# Autodesk Inventor assembly: Scoreboard
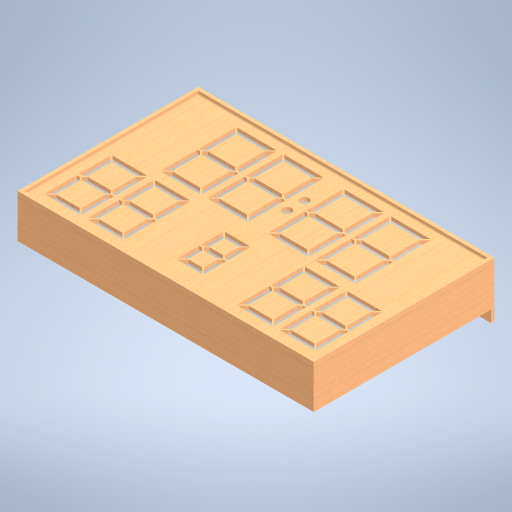
[picture p0: Inventor's stored thumbnail of the model, 512x512]
Saved by Autodesk Inventor 2024 (Build 280153000, 153)
## iProperties
Created: 2024-02-15
Part Number: Scoreboard
Document SubType Name: Assembly
Designer: haniv
Author: haniv
## Documents named in this file (8)
- C:\Users\haniv\Desktop\Unterlagen\Projekte\7_Segment_Anzeige\ScoreDisplay\CAD\Scoreboard.iam
- C:\Users\haniv\Desktop\Unterlagen\Projekte\7_Segment_Anzeige\ScoreDisplay\CAD\Components\Aluminium_Grundplatte.ipt
- C:\Users\haniv\Desktop\Unterlagen\Projekte\7_Segment_Anzeige\ScoreDisplay\CAD\Components\MDF_Anzeige.ipt
- C:\Users\haniv\Desktop\Unterlagen\Projekte\7_Segment_Anzeige\ScoreDisplay\CAD\Components\Längsseite_Gehäuse.ipt
- C:\Users\haniv\Desktop\Unterlagen\Projekte\7_Segment_Anzeige\ScoreDisplay\CAD\Components\Querseite_Gehäuse.ipt
- C:\Users\haniv\Desktop\Unterlagen\Projekte\7_Segment_Anzeige\ScoreDisplay\CAD\Components\Oberseite_Gehäuse.ipt
- C:\Users\haniv\Desktop\Unterlagen\Projekte\7_Segment_Anzeige\ScoreDisplay\CAD\Components\Gummidichtung.ipt
- C:\Users\haniv\Desktop\Unterlagen\Projekte\7_Segment_Anzeige\ScoreDisplay\CAD\Components\Rückseite_Gehäuse.ipt
## Components (8 placed, 7 different names)
1. Aluminium_Grundplatte:1 — Passend:1, Fluchtend:1, Fluchtend:2
2. MDF_Anzeige:1 — Passend:1, Fluchtend:1, Fluchtend:2, Passend:3, Passend:6, Passend:9, Fluchtend:8
3. Querseite_Gehäuse:1 — Passend:3, Passend:10, Fluchtend:10, Fluchtend:12, Passend:13, Tangential:1, Fluchtend:14
4. Querseite_Gehäuse:2 — Passend:6, Passend:8, Fluchtend:6, Fluchtend:7, Passend:11, Fluchtend:11, Fluchtend:13, Tangential:2
5. Längsseite_Gehäuse:2 — Passend:8, Fluchtend:6, Fluchtend:7
6. Oberseite_Gehäuse:1 — Passend:9, Fluchtend:8, Passend:10, Fluchtend:10, Passend:11, Fluchtend:11, Fluchtend:12, Fluchtend:13, Passend:12, Passend:14
7. Gummidichtung:1 — Passend:12, Passend:13, Tangential:1, Tangential:2, Tangential:3
8. Rückseite_Gehäuse:1 — Passend:14, Fluchtend:14, Tangential:3
## Relationships (23: Mate 10, Flush 10, Tangent 3)
- Passend:1 [Mate]: Aluminium_Grundplatte:1 ↔ MDF_Anzeige:1
- Fluchtend:1 [Flush]: Aluminium_Grundplatte:1 ↔ MDF_Anzeige:1
- Fluchtend:2 [Flush]: Aluminium_Grundplatte:1 ↔ MDF_Anzeige:1
- Passend:3 [Mate] (1 mm): MDF_Anzeige:1 ↔ Querseite_Gehäuse:1
- Passend:6 [Mate] (1 mm): MDF_Anzeige:1 ↔ Querseite_Gehäuse:2
- Passend:8 [Mate]: Querseite_Gehäuse:2 ↔ Längsseite_Gehäuse:2
- Fluchtend:6 [Flush]: Querseite_Gehäuse:2 ↔ Längsseite_Gehäuse:2
- Fluchtend:7 [Flush]: Querseite_Gehäuse:2 ↔ Längsseite_Gehäuse:2
- Passend:9 [Mate] (1 mm): MDF_Anzeige:1 ↔ Oberseite_Gehäuse:1
- Fluchtend:8 [Flush]: MDF_Anzeige:1 ↔ Oberseite_Gehäuse:1
- Passend:10 [Mate]: Querseite_Gehäuse:1 ↔ Oberseite_Gehäuse:1
- Fluchtend:10 [Flush]: Querseite_Gehäuse:1 ↔ Oberseite_Gehäuse:1
- Passend:11 [Mate]: Querseite_Gehäuse:2 ↔ Oberseite_Gehäuse:1
- Fluchtend:11 [Flush]: Querseite_Gehäuse:2 ↔ Oberseite_Gehäuse:1
- Fluchtend:12 [Flush]: Querseite_Gehäuse:1 ↔ Oberseite_Gehäuse:1
- Fluchtend:13 [Flush]: Querseite_Gehäuse:2 ↔ Oberseite_Gehäuse:1
- Passend:12 [Mate]: Oberseite_Gehäuse:1 ↔ Gummidichtung:1
- Passend:13 [Mate]: Querseite_Gehäuse:1 ↔ Gummidichtung:1
- Tangential:1: Querseite_Gehäuse:1 ↔ Gummidichtung:1
- Tangential:2: Querseite_Gehäuse:2 ↔ Gummidichtung:1
- Passend:14 [Mate]: Oberseite_Gehäuse:1 ↔ Rückseite_Gehäuse:1
- Fluchtend:14 [Flush]: Querseite_Gehäuse:1 ↔ Rückseite_Gehäuse:1
- Tangential:3: Gummidichtung:1 ↔ Rückseite_Gehäuse:1
